# Autodesk Inventor assembly: Mounting
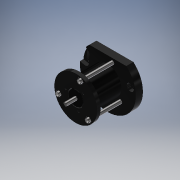
[picture p0: Inventor's stored thumbnail of the model, 180x180]
Saved by Autodesk Inventor 2018 (Build 220112000, 112)
## iProperties
Created: 2018-03-20
Part Number: Mounting
Document SubType Name: Assembly
Designer: P301319
Author: P301319
## Documents named in this file (6)
- C:\Users\P301319\Documents\GitHub\CNC-Lathe-CAD\CNC Lathe Project\Project Files\Encoder Subassembly\Mounting.iam
- C:\Users\P301319\Documents\GitHub\CNC-Lathe-CAD\CNC Lathe Project\Project Files\Encoder Subassembly\Working Encoder.iam
- C:\Users\P301319\Documents\GitHub\CNC-Lathe-CAD\CNC Lathe Project\Project Files\Encoder Subassembly\Encoder Mount Front.ipt
- C:\Users\P301319\Documents\GitHub\CNC-Lathe-CAD\CNC Lathe Project\Project Files\Encoder Subassembly\Encoder Mount Base.ipt
- C:\Users\P301319\Documents\GitHub\CNC-Lathe-CAD\CNC Lathe Project\Project Files\Encoder Subassembly\Bolt Cover.ipt
- C:\Users\P301319\Documents\GitHub\CNC-Lathe-CAD\CNC Lathe Project\Project Files\Encoder Subassembly\New Bolt.ipt
## Components (9 placed, 5 different names)
1. Working Encoder:1 [sub-assembly] — Mate:1, Mate:7, Mate:9, Mate:11
2. Encoder Mount Base:1 — Mate:1, Mate:4, Mate:6, Mate:10, Angle:1, Mate:24, Mate:25
3. Encoder Mount Front:1 — Mate:7, Mate:9, Mate:11, Mate:12, Mate:13, Mate:14, Mate:15, Mate:16, Mate:17, Mate:21, Mate:22, Mate:23
4. Bolt Cover:1 — Mate:18, Mate:22
5. Bolt Cover:2 — Mate:19, Mate:23
6. Bolt Cover:3 — Mate:20, Mate:21, Mate:25
7. New Bolt:1 — Mate:12, Mate:16, Mate:19
8. New Bolt:2 — Mate:13, Mate:17, Mate:18
9. New Bolt:3 — Mate:14, Mate:15, Mate:20, Mate:24
## Relationships (22: Mate 21, Angle 1)
- Mate:1: Working Encoder:1 ↔ Encoder Mount Base:1
- Mate:4: Encoder Mount Base:1
- Mate:6: Encoder Mount Base:1
- Mate:7: Working Encoder:1 ↔ Encoder Mount Front:1
- Mate:9: Working Encoder:1 ↔ Encoder Mount Front:1
- Mate:10: Encoder Mount Base:1
- Angle:1 (0 deg): Encoder Mount Base:1
- Mate:11: Working Encoder:1 ↔ Encoder Mount Front:1
- Mate:12: Encoder Mount Front:1 ↔ New Bolt:1
- Mate:13: Encoder Mount Front:1 ↔ New Bolt:2
- Mate:14: Encoder Mount Front:1 ↔ New Bolt:3
- Mate:15: Encoder Mount Front:1 ↔ New Bolt:3
- Mate:16: Encoder Mount Front:1 ↔ New Bolt:1
- Mate:17: Encoder Mount Front:1 ↔ New Bolt:2
- Mate:18: Bolt Cover:1 ↔ New Bolt:2
- Mate:19: Bolt Cover:2 ↔ New Bolt:1
- Mate:20: Bolt Cover:3 ↔ New Bolt:3
- Mate:21: Encoder Mount Front:1 ↔ Bolt Cover:3
- Mate:22: Encoder Mount Front:1 ↔ Bolt Cover:1
- Mate:23: Encoder Mount Front:1 ↔ Bolt Cover:2
- Mate:24: Encoder Mount Base:1 ↔ New Bolt:3
- Mate:25: Encoder Mount Base:1 ↔ Bolt Cover:3
